# Autodesk Inventor assembly: Timing_Assy_Lever Shaft 2 Lanes
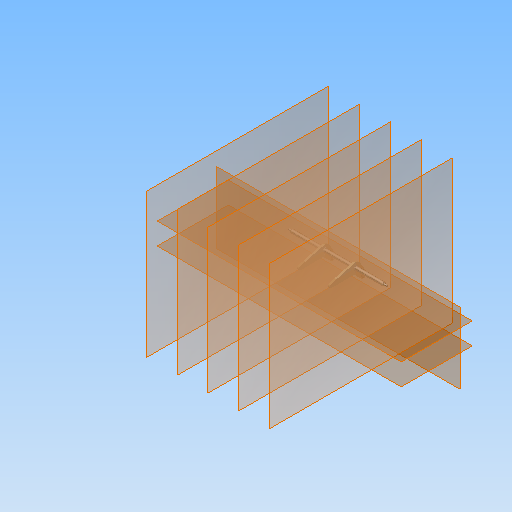
[picture p0: Inventor's stored thumbnail of the model, 512x512]
Saved by Autodesk Inventor 2018.1 (Build 221171000, 171)
## iProperties
Created: 2019-02-11
Part Number: Timing_Assy_Lever Shaft 2 Lanes
Document SubType Name: Assembly
Designer: James
Author: James
## Documents named in this file (7)
- C:\Users\admin\Desktop\Ball Sorting Machine\Ball-Sorting-Machine\Timing Gate\Timing - 2 Lanes\Timing_Assy_Lever Shaft 2 Lanes.iam
- C:\Users\admin\Desktop\Ball Sorting Machine\Ball-Sorting-Machine\Timing Gate\Timing_Lever.ipt
- C:\Users\admin\Desktop\Ball Sorting Machine\Ball-Sorting-Machine\Timing Gate\Timing_Lever Weight.ipt
- C:\Users\admin\Desktop\Ball Sorting Machine\Ball-Sorting-Machine\Timing Gate\BS 3673 - 6mm External Circlip.ipt
- C:\Users\admin\Desktop\Ball Sorting Machine\Ball-Sorting-Machine\Timing Gate\M3 x 0.5mm Zinc Plated Steel Washer.ipt
- C:\Users\admin\Desktop\Ball Sorting Machine\Ball-Sorting-Machine\Timing Gate\Socket Button Head - (A2) - M3 x 10.ipt
- C:\Users\admin\Desktop\Ball Sorting Machine\Ball-Sorting-Machine\Timing Gate\Timing - 2 Lanes\Timing_Lever Shaft 2 Lanes.ipt
## Components (13 placed, 6 different names)
1. Timing_Lever:1 — Mate:6, Mate:7, Mate:8, Flush:9, Mate:13, Mate:14, Mate:16
2. Timing_Lever Shaft 2 Lanes:1 — Flush:8, Mate:6, Flush:9, Mate:9, Mate:10, Mate:11, Mate:12, Mate:41, Flush:16, Flush:17
3. Timing_Lever Weight:1 — Mate:7, Mate:8
4. M3 x 0.5mm Zinc Plated Steel Washer:1 — Mate:13, Mate:14, Mate:15
5. Socket Button Head - (A2) - M3 x 10:1 — Mate:15, Mate:16
6. Timing_Lever:2 — Mate:41, Mate:48
7. Timing_Lever Weight:2
8. M3 x 0.5mm Zinc Plated Steel Washer:2
9. Socket Button Head - (A2) - M3 x 10:2
10. BS 3673 - 6mm External Circlip:2 — Mate:9, Mate:12, Flush:10, Angle:2
11. BS 3673 - 6mm External Circlip:1 — Mate:10, Mate:11, Flush:10
12. BS 3673 - 6mm External Circlip:3 — Mate:48
13. BS 3673 - 6mm External Circlip:4
## Component patterns: (2 elements, first: BS 3673 - 6mm External Circlip:2 + BS 3673 - 6mm External Circlip:1)
## Relationships (28: Mate 19, Flush 8, Angle 1)
- Flush:8: Timing_Lever Shaft 2 Lanes:1
- Mate:6: Timing_Lever:1 ↔ Timing_Lever Shaft 2 Lanes:1
- Mate:7: Timing_Lever:1 ↔ Timing_Lever Weight:1
- Mate:8: Timing_Lever:1 ↔ Timing_Lever Weight:1
- Flush:9: Timing_Lever:1 ↔ Timing_Lever Shaft 2 Lanes:1
- Mate:9: Timing_Lever Shaft 2 Lanes:1 ↔ BS 3673 - 6mm External Circlip:2
- Mate:10: Timing_Lever Shaft 2 Lanes:1 ↔ BS 3673 - 6mm External Circlip:1
- Mate:11: Timing_Lever Shaft 2 Lanes:1 ↔ BS 3673 - 6mm External Circlip:1
- Mate:12: Timing_Lever Shaft 2 Lanes:1 ↔ BS 3673 - 6mm External Circlip:2
- Flush:10: BS 3673 - 6mm External Circlip:2 ↔ BS 3673 - 6mm External Circlip:1
- Angle:2 (180 deg): BS 3673 - 6mm External Circlip:2
- Mate:13: Timing_Lever:1 ↔ M3 x 0.5mm Zinc Plated Steel Washer:1
- Mate:14: Timing_Lever:1 ↔ M3 x 0.5mm Zinc Plated Steel Washer:1
- Mate:15: M3 x 0.5mm Zinc Plated Steel Washer:1 ↔ Socket Button Head - (A2) - M3 x 10:1
- Mate:16: Timing_Lever:1 ↔ Socket Button Head - (A2) - M3 x 10:1
- [Mate]: Timing_Lever:2 ↔ Timing_Lever Weight:2
- [Mate]: Timing_Lever:2 ↔ Timing_Lever Weight:2
- [Mate]: Timing_Lever:2 ↔ M3 x 0.5mm Zinc Plated Steel Washer:2
- [Mate]: Timing_Lever:2 ↔ M3 x 0.5mm Zinc Plated Steel Washer:2
- [Mate]: M3 x 0.5mm Zinc Plated Steel Washer:2 ↔ Socket Button Head - (A2) - M3 x 10:2
- [Mate]: Timing_Lever:2 ↔ Socket Button Head - (A2) - M3 x 10:2
- Mate:41: Timing_Lever Shaft 2 Lanes:1 ↔ Timing_Lever:2
- Mate:48: Timing_Lever:2 ↔ BS 3673 - 6mm External Circlip:3
- Flush:11 (-58 mm)
- Flush:12 (-5 mm)
- Flush:13 (30 mm)
- Flush:16: Timing_Lever Shaft 2 Lanes:1
- Flush:17: Timing_Lever Shaft 2 Lanes:1
## Named parameters: d37_d20 = 0 mm, d38_d21 = 0 mm, d39_d33 = 0 mm, d40_d34 = 0 mm, d41_d35 = 0 mm, d42_d36 = 0 mm
